# Autodesk Inventor assembly: ASY GBK 1120 long wall shield 2
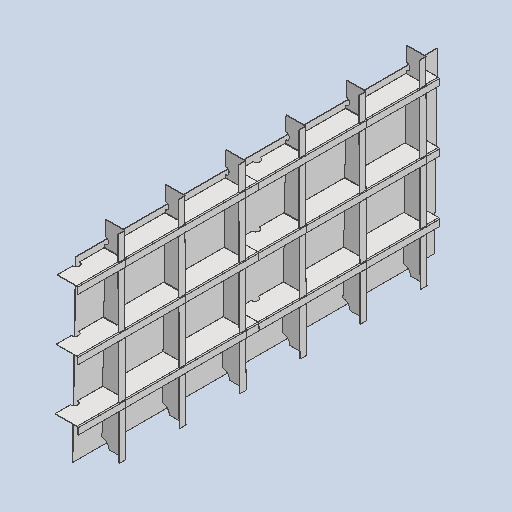
[picture p0: Inventor's stored thumbnail of the model, 512x512]
Saved by Autodesk Inventor 2026.2 (Build 302298000, 298)
## iProperties
Created: 2026-05-07
Part Number: ASY GBK 1120 long wall shield 2
Document SubType Name: Assembly
Designer: pokla
Mass: 272186 g
Surface Area: 175796 cm^2
Volume: 34673.3 cm^3
Density: 7.85 g/cm^3
Stock Number: 1112
Author: admin
## Documents named in this file (6)
- C:\Users\admin\Documents\Inventor\GBK-Gubkinskiy\ASY GBK 1120 long wall shield 2.iam
- C:\Users\admin\Documents\Inventor\GBK-Gubkinskiy\GBK 1211 shield 2.ipt
- C:\Users\admin\Documents\Inventor\GBK-Gubkinskiy\GBK 1112 stringer 1.ipt
- C:\Users\admin\Documents\Inventor\GBK-Gubkinskiy\GBK 1113 stringer 2.ipt
- C:\Users\admin\Documents\Inventor\GBK-Gubkinskiy\GBK 1114 stringer 3.ipt
- C:\Users\admin\Documents\Inventor\GBK-Gubkinskiy\GBK 1111 main rib.ipt
## Components (13 placed, 5 different names)
1. GBK 1112 stringer 1:1
2. GBK 1112 stringer 1:2
3. GBK 1113 stringer 2:1
4. GBK 1113 stringer 2:2
5. GBK 1114 stringer 3:1
6. GBK 1114 stringer 3:2
7. GBK 1018 shield 2:1
8. GBK 1111 main rib:1
9. GBK 1111 main rib:2
10. GBK 1111 main rib:3
11. GBK 1111 main rib:4
12. GBK 1111 main rib:5
13. GBK 1111 main rib:6
## Component patterns: (6 elements, first: GBK 1111 main rib:1)
## Relationships (9: WeldJoint 6, Mate 2, Flush 1)
- [WeldJoint]: GBK 1112 stringer 1:1 ↔ GBK 1112 stringer 1:2
- [WeldJoint]: GBK 1113 stringer 2:1 ↔ GBK 1113 stringer 2:2
- [WeldJoint]: GBK 1114 stringer 3:1 ↔ GBK 1114 stringer 3:2
- [Flush] (254 mm): GBK 1018 shield 2:1 ↔ GBK 1111 main rib:1
- [Mate]: GBK 1018 shield 2:1 ↔ GBK 1111 main rib:1
- [Mate]: GBK 1018 shield 2:1 ↔ GBK 1111 main rib:1
- [WeldJoint] (4 mm): GBK 1112 stringer 1:1 ↔ GBK 1111 main rib:1
- [WeldJoint] (4 mm): GBK 1113 stringer 2:1 ↔ GBK 1111 main rib:1
- [WeldJoint] (4 mm): GBK 1114 stringer 3:1 ↔ GBK 1111 main rib:1
## Named parameters: Шаг_шпангоутов = 496.66667 mm
